# Autodesk Inventor assembly: Door Carriage 2 Wheel
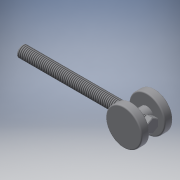
[picture p0: Inventor's stored thumbnail of the model, 180x180]
Saved by Autodesk Inventor 2016 (Build 200138000, 138)
## iProperties
Created: 2017-10-31
Part Number: Door Carriage 2 Wheel
Document SubType Name: Assembly
Designer: M227562
Author: M227562
## Documents named in this file (3)
- C:\Users\M227562\Documents\Arexu san\Door Carriage 2 Wheel.iam
- C:\Users\M227562\Documents\Arexu san\Wheels.ipt
- C:\Users\M227562\Documents\Arexu san\Rod for Wheels.ipt
## Components (2 placed, 2 different names)
1. Wheels:1 — Cylindrical:1, Mate:1
2. Rod for Wheels:1 — Cylindrical:1, Mate:1
## Relationships (2: CylindricalJoint 1, Mate 1)
- Cylindrical:1: Wheels:1 ↔ Rod for Wheels:1
- Mate:1 (6.5 mm): Wheels:1 ↔ Rod for Wheels:1
